# Autodesk Inventor assembly: Chain Drive
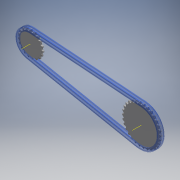
[picture p0: Inventor's stored thumbnail of the model, 180x180]
Saved by Autodesk Inventor 2019 (Build 230136000, 136)
## iProperties
ClientObjectVersion: 1
Created: 2019-11-15
Part Number: Chain Drive
Document SubType Name: Assembly
Designer: Domenico
Author: Domenico
## Documents named in this file (4)
- C:\Users\Domenico\Documents\Inventor\Mecanismos2\Robot Triciclo - Ensamble\Design Accelerator\Chain Drive1.iam
- C:\Users\Domenico\Documents\Inventor\Mecanismos2\Robot Triciclo - Ensamble\Design Accelerator\Roller Chain1.ipt
- C:\Users\Domenico\Documents\Inventor\Mecanismos2\Robot Triciclo - Ensamble\Design Accelerator\Roller Chain Sprocket11.ipt
- C:\Users\Domenico\Documents\Inventor\Mecanismos2\Robot Triciclo - Ensamble\Design Accelerator\Roller Chain Sprocket21.ipt
## Components (3 placed, 3 different names)
1. Cadena:1 — Flush:1, Mate:1, Mate:2, Flush:2, Mate:3, Mate:4
2. Sprocket1:1 — Flush:1, Mate:1, Mate:2, Rotation:1
3. Sprocket2:1 — Flush:2, Mate:3, Rotation:1, Mate:4
## Relationships (7: Mate 4, Flush 2, RelateRotation 1)
- Flush:1: Cadena:1 ↔ Sprocket1:1
- Mate:1: Cadena:1 ↔ Sprocket1:1
- Mate:2: Cadena:1 ↔ Sprocket1:1
- Flush:2: Cadena:1 ↔ Sprocket2:1
- Mate:3: Cadena:1 ↔ Sprocket2:1
- Rotation:1 [RelateRotation] (0.6333 ul): Sprocket1:1 ↔ Sprocket2:1
- Mate:4: Cadena:1 ↔ Sprocket2:1
